# Autodesk Inventor assembly: cala_przypinka
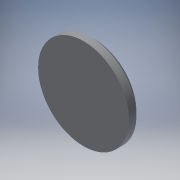
[picture p0: Inventor's stored thumbnail of the model, 180x180]
Saved by Autodesk Inventor 2019 (Build 230136000, 136)
## iProperties
Created: 2020-10-14
Part Number: cala_przypinka
Material: Ogólny
Document SubType Name: Assembly
Designer: Dawid
Author: Dawid
## Documents named in this file (6)
- C:\Users\Dawid\Downloads\cala_przypinka.iam
- C:\Users\Dawid\Downloads\przypinka.ipt
- C:\Users\Dawid\Downloads\literkaa.ipt
- C:\Users\Dawid\Downloads\literaa2.ipt
- C:\Users\Dawid\Downloads\literak.ipt
- C:\Users\Dawid\Downloads\literai.ipt
## Components (5 placed, 5 different names)
1. przypinka:1 — Równoległy:1
2. literkaa:1
3. literaa2:1
4. literak:1 — Równoległy:1
5. literai:1
## Relationships (1: Flush 1)
- Równoległy:1 [Flush]: przypinka:1 ↔ literak:1
